# Autodesk Inventor assembly: Outer
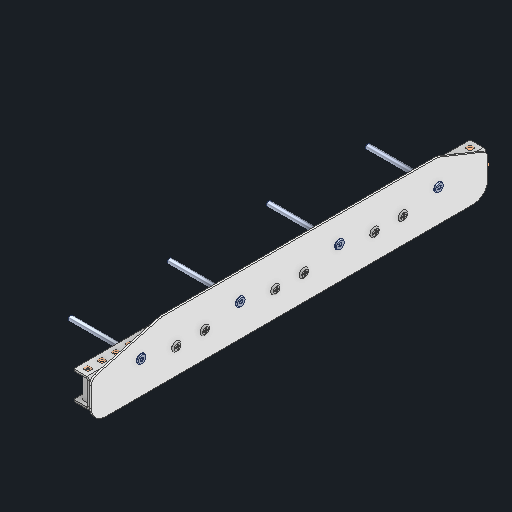
[picture p0: Inventor's stored thumbnail of the model, 512x512]
Saved by Autodesk Inventor 2025 (Build 290162000, 162)
## iProperties
Created: 2024-12-17
Part Number: Outer
Document SubType Name: Assembly
Designer: avere
Author: avere
## Documents named in this file (10)
- D:\VEX\High Stakes\CAD\V4\Chassis\Drivebay Left\Outer.iam
- D:\VEX\High Stakes\CAD\ROBOPROS-CAD-Inventor\Structure\C Channel\Aluminum 1x2x1\Alu C 1x2x1x28.ipt
- D:\VEX\High Stakes\CAD\V4\Chassis\Drivebay Left\Custom Parts\Skirt.ipt
- D:\VEX\High Stakes\CAD\ROBOPROS-CAD-Inventor\Structure\Hardware\Screw Steel - Star\SScrew Star Smooth 2.500.ipt
- D:\VEX\High Stakes\CAD\ROBOPROS-CAD-Inventor\Structure\Hardware\Screw Steel - Star.ipt
- D:\VEX\High Stakes\CAD\ROBOPROS-CAD-Inventor\Structure\Hardware\Nut Keps.ipt
- D:\VEX\High Stakes\CAD\ROBOPROS-CAD-Inventor\Structure\Hardware\Screw Nylon - Pan Head\NScrew Pan Head Threaded .500.ipt
- D:\VEX\High Stakes\CAD\ROBOPROS-CAD-Inventor\Structure\Hardware\Nut Nylon Thread-Forming.ipt
- D:\VEX\High Stakes\CAD\ROBOPROS-CAD-Inventor\Motion\Shaft LS\Bearing Flat Low Profile.ipt
- D:\VEX\High Stakes\CAD\ROBOPROS-CAD-Inventor\Structure\Nylon Standoff Rounded\Nylon Standoff .875.ipt
## Components (26 placed, 8 different names)
1. Alu C 1x2x1x28:1 — Flush:1, Flush:2, Flush:3, Insert:1, Mate:1, Insert:3, Insert:8, Mate:2, Insert:9
2. Skirt:1 — Insert:1, Mate:1, Insert:2, Insert:4, Insert:5
3. Nylon Standoff .875:1 — Insert:9
4. Nut Keps:1 — Insert:3
5. SScrew Star Smooth 2.500:1 — Insert:2
6. Nut Keps:2
7. SScrew Star Smooth 2.500:2
8. Nut Keps:3
9. SScrew Star Smooth 2.500:3
10. Nut Keps:4
11. SScrew Star Smooth 2.500:4
12. Bearing Flat Low Profile:1 — Insert:6, Insert:7, Insert:8, Mate:2
13. Nut Nylon Thread-Forming:2 — Insert:7
14. Nut Nylon Thread-Forming:1 — Insert:6
15. NScrew Pan Head Threaded .500:2 — Insert:5
16. NScrew Pan Head Threaded .500:1 — Insert:4
17. Bearing Flat Low Profile:2
18. Nut Nylon Thread-Forming:3
19. Nut Nylon Thread-Forming:4
20. NScrew Pan Head Threaded .500:3
21. NScrew Pan Head Threaded .500:4
22. Bearing Flat Low Profile:3
23. Nut Nylon Thread-Forming:5
24. Nut Nylon Thread-Forming:6
25. NScrew Pan Head Threaded .500:5
26. NScrew Pan Head Threaded .500:6
## Component patterns: Screw Joints (4 elements), Bearings (3 elements)
## Relationships (14: Insert 9, Flush 3, Mate 2)
- Flush:1 (-177.8 mm): Alu C 1x2x1x28:1
- Flush:2 (-12.7 mm): Alu C 1x2x1x28:1
- Flush:3 (-7.9375 mm): Alu C 1x2x1x28:1
- Insert:1: Alu C 1x2x1x28:1 ↔ Skirt:1
- Mate:1: Alu C 1x2x1x28:1 ↔ Skirt:1
- Insert:2: Skirt:1 ↔ SScrew Star Smooth 2.500:1
- Insert:3: Alu C 1x2x1x28:1 ↔ Nut Keps:1
- Insert:4 (-1.5875 mm): Skirt:1 ↔ NScrew Pan Head Threaded .500:1
- Insert:5 (-1.5875 mm): Skirt:1 ↔ NScrew Pan Head Threaded .500:2
- Insert:6 (1.27 mm): Bearing Flat Low Profile:1 ↔ Nut Nylon Thread-Forming:1
- Insert:7 (1.27 mm): Bearing Flat Low Profile:1 ↔ Nut Nylon Thread-Forming:2
- Insert:8: Alu C 1x2x1x28:1 ↔ Bearing Flat Low Profile:1
- Mate:2: Alu C 1x2x1x28:1 ↔ Bearing Flat Low Profile:1
- Insert:9: Alu C 1x2x1x28:1 ↔ Nylon Standoff .875:1
